# Autodesk Inventor assembly: Counter2
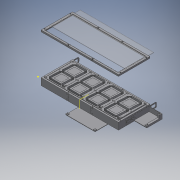
[picture p0: Inventor's stored thumbnail of the model, 180x180]
Saved by Autodesk Inventor 2016 SP2 (Build 200236200, 236)
## iProperties
Created: 2018-06-10
Part Number: Counter2
Material: Generisch
Document SubType Name: Assembly
Designer: Nils
Author: Nils
## Documents named in this file (20)
- C:\Users\Nils\Documents\Projects\Big Stopwatch\Big-Stopwatch\Models\Counter\Counter2.iam
- C:\Users\Nils\Documents\Projects\Big Stopwatch\Big-Stopwatch\Models\Counter\Scheibe.ipt
- C:\Users\Nils\Documents\Projects\Big Stopwatch\Big-Stopwatch\Models\Counter\Backplate-housing.ipt
- C:\Users\Nils\Documents\Projects\Big Stopwatch\Big-Stopwatch\Models\Counter\Zwischenplatt.ipt
- C:\Users\Nils\Documents\Projects\Big Stopwatch\Big-Stopwatch\Models\Counter\Knopf.ipt
- C:\Users\Nils\Documents\Projects\Big Stopwatch\Big-Stopwatch\Models\Counter\Case-Side.ipt
- C:\Users\Nils\Documents\Projects\Big Stopwatch\Big-Stopwatch\Models\Counter\Case_side_back.ipt
- C:\Users\Nils\Documents\Projects\Big Stopwatch\Big-Stopwatch\Models\Counter\Case_bottom_front.ipt
- C:\Users\Nils\Documents\Projects\Big Stopwatch\Big-Stopwatch\Models\Counter\Case_bottom_back.ipt
- C:\Users\Nils\Documents\Projects\Big Stopwatch\Big-Stopwatch\Models\Counter\Case_top_back.ipt
- C:\Users\Nils\Documents\Projects\Big Stopwatch\Big-Stopwatch\Models\Counter\Case-Side_MIR.ipt
- C:\Users\Nils\Documents\Projects\Big Stopwatch\Big-Stopwatch\Models\Counter\Case_side_back_MIR1.ipt
- C:\Users\Nils\Documents\Projects\Big Stopwatch\Big-Stopwatch\Models\Counter\Batcap3.ipt
- C:\Users\Nils\Documents\Projects\Big Stopwatch\Big-Stopwatch\Models\Counter\Batcap3_MIR.ipt
- C:\Users\Nils\Documents\Projects\Big Stopwatch\Big-Stopwatch\Models\Counter\PCB-Mount.ipt
- C:\Users\Nils\Documents\Projects\Big Stopwatch\Big-Stopwatch\Models\Counter\Screw-right.ipt
- C:\Users\Nils\Documents\Projects\Big Stopwatch\Big-Stopwatch\Models\Counter\Screw-left.ipt
- C:\Users\Nils\Documents\Projects\Big Stopwatch\Big-Stopwatch\Models\Counter\hangmount.ipt
- C:\Users\Nils\Documents\Projects\Big Stopwatch\Big-Stopwatch\Models\Counter\Zwischenplatt_MIR.ipt
- C:\Users\Nils\Documents\Projects\Big Stopwatch\Big-Stopwatch\Models\Counter\Digit.iam
## Components (31 placed, 19 different names)
1. Scheibe:1 — Passend:52, Passend:53
2. Case-Side:1 — Fluchtend:60, Fluchtend:61, Passend:52, Passend:53
3. Case_side_back:1 — Fluchtend:45, Fluchtend:46, Fluchtend:48, Fluchtend:49, Passend:36, Passend:40, Passend:41, Passend:45, Fluchtend:55, Fluchtend:56, Passend:54
4. Case_bottom_front:1 — Fluchtend:37
5. Case_bottom_back:1 — Passend:51
6. Zwischenplatt:1
7. Backplate-housing:1
8. Case_bottom_front:2 — Fluchtend:37, Fluchtend:60, Fluchtend:61, Fluchtend:62, Fluchtend:63, Passend:47
9. Case_top_back:1 — Passend:35
10. Case-Side_MIR:1 — Fluchtend:62, Fluchtend:63, Passend:47
11. Case_side_back_MIR1:1 — Fluchtend:45, Fluchtend:46, Passend:35, Fluchtend:50, Fluchtend:51, Passend:37, Passend:44, Passend:46, Passend:48, Passend:49, Passend:50
12. Batcap3:1 — Fluchtend:48, Fluchtend:49, Passend:36
13. Batcap3_MIR:1 — Fluchtend:50, Fluchtend:51, Passend:37
14. PCB-Mount:1
15. Zwischenplatt_MIR:1 — Passend:48, Passend:49, Passend:50
16. Screw-right:1 — Passend:40, Fluchtend:53, Passend:43
17. Screw-right:2 — Passend:41, Fluchtend:53, Passend:42, Passend:45
18. Screw-left:1 — Fluchtend:54, Passend:43
19. Screw-left:2 — Fluchtend:54, Passend:42, Passend:44
20. hangmount:1 — Fluchtend:55, Fluchtend:56, Fluchtend:57, Fluchtend:58
21. hangmount:2 — Passend:46, Fluchtend:57, Fluchtend:58
22. Knopf:1
23. Knopf:2
24. Knopf:3
25. Knopf:4
26. Knopf:5
27. Knopf:6
28. Digit:1 [sub-assembly] — Passend:54
29. Digit:2 [sub-assembly] — Passend:51
30. Digit:3 [sub-assembly]
31. Digit:4 [sub-assembly]
## Component patterns: (6 elements, first: Knopf:1), (4 elements, first: Digit:1)
## Relationships (35: Mate 18, Flush 17)
- Fluchtend:37 [Flush]: Case_bottom_front:1 ↔ Case_bottom_front:2
- Fluchtend:45 [Flush]: Case_side_back:1 ↔ Case_side_back_MIR1:1
- Fluchtend:46 [Flush]: Case_side_back:1 ↔ Case_side_back_MIR1:1
- Passend:35 [Mate] (0.1 mm): Case_top_back:1 ↔ Case_side_back_MIR1:1
- Fluchtend:48 [Flush]: Case_side_back:1 ↔ Batcap3:1
- Fluchtend:49 [Flush]: Case_side_back:1 ↔ Batcap3:1
- Passend:36 [Mate] (211.248 mm): Case_side_back:1 ↔ Batcap3:1
- Fluchtend:50 [Flush]: Case_side_back_MIR1:1 ↔ Batcap3_MIR:1
- Fluchtend:51 [Flush]: Case_side_back_MIR1:1 ↔ Batcap3_MIR:1
- Passend:37 [Mate] (270.899 mm): Case_side_back_MIR1:1 ↔ Batcap3_MIR:1
- Passend:40 [Mate]: Case_side_back:1 ↔ Screw-right:1
- Passend:41 [Mate]: Case_side_back:1 ↔ Screw-right:2
- Fluchtend:53 [Flush]: Screw-right:1 ↔ Screw-right:2
- Fluchtend:54 [Flush]: Screw-left:1 ↔ Screw-left:2
- Passend:42 [Mate]: Screw-right:2 ↔ Screw-left:2
- Passend:43 [Mate]: Screw-right:1 ↔ Screw-left:1
- Passend:44 [Mate] (-3 mm): Case_side_back_MIR1:1 ↔ Screw-left:2
- Passend:45 [Mate] (-3 mm): Case_side_back:1 ↔ Screw-right:2
- Fluchtend:55 [Flush]: Case_side_back:1 ↔ hangmount:1
- Fluchtend:56 [Flush]: Case_side_back:1 ↔ hangmount:1
- Passend:46 [Mate]: Case_side_back_MIR1:1 ↔ hangmount:2
- Fluchtend:57 [Flush]: hangmount:1 ↔ hangmount:2
- Fluchtend:58 [Flush]: hangmount:1 ↔ hangmount:2
- Fluchtend:60 [Flush]: Case-Side:1 ↔ Case_bottom_front:2
- Fluchtend:61 [Flush]: Case-Side:1 ↔ Case_bottom_front:2
- Fluchtend:62 [Flush]: Case_bottom_front:2 ↔ Case-Side_MIR:1
- Fluchtend:63 [Flush]: Case_bottom_front:2 ↔ Case-Side_MIR:1
- Passend:47 [Mate]: Case_bottom_front:2 ↔ Case-Side_MIR:1
- Passend:48 [Mate] (0.1 mm): Case_side_back_MIR1:1 ↔ Zwischenplatt_MIR:1
- Passend:49 [Mate] (0.1 mm): Case_side_back_MIR1:1 ↔ Zwischenplatt_MIR:1
- Passend:50 [Mate] (0.1 mm): Case_side_back_MIR1:1 ↔ Zwischenplatt_MIR:1
- Passend:51 [Mate] (0.2 mm): Case_bottom_back:1 ↔ Digit:2
- Passend:52 [Mate]: Scheibe:1 ↔ Case-Side:1
- Passend:53 [Mate] (2 mm): Scheibe:1 ↔ Case-Side:1
- Passend:54 [Mate] (2.5 mm): Case_side_back:1 ↔ Digit:1
